# Autodesk Inventor assembly: electronics
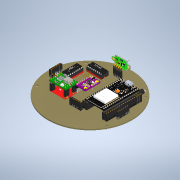
[picture p0: Inventor's stored thumbnail of the model, 180x180]
Saved by Autodesk Inventor 2020.2 (Build 242310000, 310)
## iProperties
Created: 2020-06-15
Part Number: electronics
Document SubType Name: Assembly
Designer: Tarsoly
Author: Tarsoly
## Documents named in this file (16)
- D:\Users\Tarsoly\Dokumentumok\BME\8. Félév\Önlab\3d\electronics.iam
- D:\Users\Tarsoly\Dokumentumok\BME\8. Félév\Önlab\3d\pins\socket\10x1\FH01-10SS.iam
- D:\Users\Tarsoly\Dokumentumok\BME\8. Félév\Önlab\3d\pins\socket\9x1\FH01-09SS.iam
- D:\Users\Tarsoly\Dokumentumok\BME\8. Félév\Önlab\3d\ESP32\ESP32S Dev Board 0.9inch width ASSY_TOP.iam
- D:\Users\Tarsoly\Dokumentumok\BME\8. Félév\Önlab\3d\PCB_v2\main_board.iam
- D:\Users\Tarsoly\Dokumentumok\BME\8. Félév\Önlab\3d\pins\socket\6x1\FH01-06SS.iam
- D:\Users\Tarsoly\Dokumentumok\BME\8. Félév\Önlab\3d\pins\dip_socket\IC_Sockel_16P.ipt
- D:\Users\Tarsoly\Dokumentumok\BME\8. Félév\Önlab\3d\L293D\L293D v1.iam
- D:\Users\Tarsoly\Dokumentumok\BME\8. Félév\Önlab\3d\pins\socket\4x1\FH01-04SS.iam
- D:\Users\Tarsoly\Dokumentumok\BME\8. Félév\Önlab\3d\pins\socket\3x1\FH01-03SS.iam
- D:\Users\Tarsoly\Dokumentumok\BME\8. Félév\Önlab\3d\pins\socket\2x1\FH01-02SS.iam
- D:\Users\Tarsoly\Dokumentumok\BME\8. Félév\Önlab\3d\pins\header\Pin Header 1x2 TH Pitch 2.54mm.ipt
- D:\Users\Tarsoly\Dokumentumok\BME\8. Félév\Önlab\3d\pins\header\Pin Header 1x4 TH Angle Pitch 2.54mm.ipt
- D:\Users\Tarsoly\Dokumentumok\BME\8. Félév\Önlab\3d\MPU2950\GY-91.iam
- D:\Users\Tarsoly\Dokumentumok\BME\8. Félév\Önlab\3d\VL5310X\vl53l0x.ipt
- D:\Users\Tarsoly\Dokumentumok\BME\8. Félév\Önlab\3d\DSN-1504\DC-DC 4.5-28V to 0.8-20V Output 3A MP1584EN Step Down Buck Converter_TOP.iam
## Components (32 placed, 15 different names)
1. FH01-10SS:1 [sub-assembly]
2. FH01-10SS:2 [sub-assembly]
3. FH01-09SS:1 [sub-assembly]
4. FH01-09SS:2 [sub-assembly]
5. ESP32S Dev Board 0.9inch width ASSY_TOP:1 [sub-assembly]
6. main_board:1 [sub-assembly]
7. FH01-10SS:3 [sub-assembly]
8. FH01-09SS:3 [sub-assembly]
9. FH01-10SS:4 [sub-assembly]
10. FH01-09SS:4 [sub-assembly]
11. FH01-06SS:1 [sub-assembly]
12. FH01-06SS:2 [sub-assembly]
13. FH01-06SS:3 [sub-assembly]
14. IC_Sockel_16P:1
15. IC_Sockel_16P:2
16. L293D v1:1 [sub-assembly]
17. L293D v1:2 [sub-assembly]
18. FH01-04SS:1 [sub-assembly]
19. FH01-04SS:2 [sub-assembly]
20. FH01-03SS:1 [sub-assembly]
21. FH01-02SS:1 [sub-assembly]
22. FH01-02SS:2 [sub-assembly]
23. Pin Header 1x2 TH Pitch 2.54mm:1
24. Pin Header 1x2 TH Pitch 2.54mm:2
25. Pin Header 1x4 TH Angle Pitch 2.54mm:1
26. FH01-02SS:3 [sub-assembly]
27. FH01-02SS:4 [sub-assembly]
28. GY-91:1 [sub-assembly]
29. vl53l0x:1
30. DC-DC 4.5-28V to 0.8-20V Output 3A MP1584EN Step Down Buck Converter_TOP:1 [sub-assembly]
31. Pin Header 1x2 TH Pitch 2.54mm:3
32. Pin Header 1x2 TH Pitch 2.54mm:4
## Relationships (87: Mate 77, Flush 8, Angle 2)
- [Mate]: FH01-09SS:1 ↔ ESP32S Dev Board 0.9inch width ASSY_TOP:1
- [Flush]: FH01-09SS:2 ↔ ESP32S Dev Board 0.9inch width ASSY_TOP:1
- [Flush]: FH01-09SS:2 ↔ ESP32S Dev Board 0.9inch width ASSY_TOP:1
- [Mate]: FH01-09SS:1 ↔ main_board:1
- [Mate]: FH01-09SS:1 ↔ main_board:1
- [Mate]: FH01-10SS:1 ↔ main_board:1
- [Mate]: FH01-10SS:1 ↔ main_board:1
- [Mate]: FH01-09SS:2 ↔ main_board:1
- [Mate]: FH01-09SS:2 ↔ main_board:1
- [Mate]: FH01-10SS:2 ↔ main_board:1
- [Mate]: FH01-10SS:2 ↔ main_board:1
- [Mate]: main_board:1 ↔ FH01-10SS:3
- [Mate]: main_board:1 ↔ FH01-10SS:3
- [Mate]: main_board:1 ↔ FH01-10SS:3
- [Mate]: main_board:1 ↔ FH01-09SS:3
- [Mate]: main_board:1 ↔ FH01-09SS:3
- [Mate]: main_board:1 ↔ FH01-09SS:3
- [Mate]: main_board:1 ↔ FH01-09SS:4
- [Mate]: main_board:1 ↔ FH01-09SS:4
- [Mate]: main_board:1 ↔ FH01-09SS:4
- [Mate]: main_board:1 ↔ FH01-10SS:4
- [Mate]: main_board:1 ↔ FH01-10SS:4
- [Mate]: main_board:1 ↔ FH01-10SS:4
- [Mate]: main_board:1 ↔ FH01-06SS:1
- [Mate]: main_board:1 ↔ FH01-06SS:1
- [Mate]: main_board:1 ↔ FH01-06SS:1
- [Mate]: main_board:1 ↔ FH01-06SS:2
- [Mate]: main_board:1 ↔ FH01-06SS:2
- [Mate]: main_board:1 ↔ FH01-06SS:2
- [Mate]: main_board:1 ↔ FH01-06SS:3
- [Mate]: main_board:1 ↔ FH01-06SS:3
- [Mate]: main_board:1 ↔ FH01-06SS:3
- [Mate]: main_board:1 ↔ IC_Sockel_16P:1
- [Mate]: main_board:1 ↔ IC_Sockel_16P:1
- [Mate]: main_board:1 ↔ IC_Sockel_16P:1
- [Mate]: main_board:1 ↔ IC_Sockel_16P:2
- [Mate]: main_board:1 ↔ IC_Sockel_16P:2
- [Mate]: main_board:1 ↔ IC_Sockel_16P:2
- [Mate]: IC_Sockel_16P:1 ↔ L293D v1:1
- [Mate]: IC_Sockel_16P:1 ↔ L293D v1:1
- [Mate] (-1.522 mm): IC_Sockel_16P:1 ↔ L293D v1:1
- [Mate]: IC_Sockel_16P:2 ↔ L293D v1:2
- [Mate]: IC_Sockel_16P:2 ↔ L293D v1:2
- [Mate] (-1.518 mm): IC_Sockel_16P:2 ↔ L293D v1:2
- [Mate]: main_board:1 ↔ FH01-04SS:1
- [Mate]: main_board:1 ↔ FH01-04SS:1
- [Mate]: main_board:1 ↔ FH01-04SS:1
- [Mate]: main_board:1 ↔ FH01-04SS:2
- [Mate]: main_board:1 ↔ FH01-04SS:2
- [Mate]: main_board:1 ↔ FH01-04SS:2
- [Mate]: main_board:1 ↔ FH01-03SS:1
- [Mate]: main_board:1 ↔ FH01-03SS:1
- [Mate]: main_board:1 ↔ FH01-03SS:1
- [Mate]: main_board:1 ↔ FH01-02SS:2
- [Mate]: main_board:1 ↔ FH01-02SS:1
- [Mate]: main_board:1 ↔ FH01-02SS:1
- [Mate]: main_board:1 ↔ FH01-02SS:1
- [Mate]: main_board:1 ↔ FH01-02SS:2
- [Mate]: main_board:1 ↔ FH01-02SS:2
- [Mate]: main_board:1 ↔ Pin Header 1x2 TH Pitch 2.54mm:2
- [Mate]: main_board:1 ↔ Pin Header 1x2 TH Pitch 2.54mm:1
- [Mate]: main_board:1 ↔ Pin Header 1x2 TH Pitch 2.54mm:2
- [Mate]: main_board:1 ↔ Pin Header 1x2 TH Pitch 2.54mm:1
- [Mate]: FH01-04SS:1 ↔ Pin Header 1x4 TH Angle Pitch 2.54mm:1
- [Mate]: FH01-04SS:1 ↔ Pin Header 1x4 TH Angle Pitch 2.54mm:1
- [Angle] (180 deg): FH01-04SS:1 ↔ Pin Header 1x4 TH Angle Pitch 2.54mm:1
- [Mate]: FH01-04SS:2 ↔ GY-91:1
- [Flush]: FH01-04SS:2 ↔ GY-91:1
- [Flush]: FH01-04SS:2 ↔ GY-91:1
- [Mate]: Pin Header 1x4 TH Angle Pitch 2.54mm:1 ↔ vl53l0x:1
- [Mate]: Pin Header 1x4 TH Angle Pitch 2.54mm:1 ↔ vl53l0x:1
- [Mate] (11.12 mm): main_board:1 ↔ vl53l0x:1
- [Mate]: FH01-02SS:4 ↔ DC-DC 4.5-28V to 0.8-20V Output 3A MP1584EN Step Down Buck Converter_TOP:1
- [Mate]: FH01-02SS:3 ↔ DC-DC 4.5-28V to 0.8-20V Output 3A MP1584EN Step Down Buck Converter_TOP:1
- [Mate]: FH01-02SS:4 ↔ DC-DC 4.5-28V to 0.8-20V Output 3A MP1584EN Step Down Buck Converter_TOP:1
- [Mate]: FH01-02SS:3 ↔ DC-DC 4.5-28V to 0.8-20V Output 3A MP1584EN Step Down Buck Converter_TOP:1
- [Flush] (0.55 mm): FH01-02SS:3 ↔ DC-DC 4.5-28V to 0.8-20V Output 3A MP1584EN Step Down Buck Converter_TOP:1
- [Flush] (0.55 mm): FH01-02SS:4 ↔ DC-DC 4.5-28V to 0.8-20V Output 3A MP1584EN Step Down Buck Converter_TOP:1
- [Mate]: DC-DC 4.5-28V to 0.8-20V Output 3A MP1584EN Step Down Buck Converter_TOP:1 ↔ Pin Header 1x2 TH Pitch 2.54mm:3
- [Mate]: DC-DC 4.5-28V to 0.8-20V Output 3A MP1584EN Step Down Buck Converter_TOP:1 ↔ Pin Header 1x2 TH Pitch 2.54mm:4
- [Mate]: DC-DC 4.5-28V to 0.8-20V Output 3A MP1584EN Step Down Buck Converter_TOP:1 ↔ Pin Header 1x2 TH Pitch 2.54mm:4
- [Mate]: DC-DC 4.5-28V to 0.8-20V Output 3A MP1584EN Step Down Buck Converter_TOP:1 ↔ Pin Header 1x2 TH Pitch 2.54mm:3
- [Flush] (0.53 mm): DC-DC 4.5-28V to 0.8-20V Output 3A MP1584EN Step Down Buck Converter_TOP:1 ↔ Pin Header 1x2 TH Pitch 2.54mm:3
- [Flush] (0.53 mm): DC-DC 4.5-28V to 0.8-20V Output 3A MP1584EN Step Down Buck Converter_TOP:1 ↔ Pin Header 1x2 TH Pitch 2.54mm:4
- [Mate]: FH01-02SS:2 ↔ Pin Header 1x2 TH Pitch 2.54mm:4
- [Mate]: FH01-02SS:2 ↔ Pin Header 1x2 TH Pitch 2.54mm:3
- [Angle] (180 deg): FH01-02SS:2 ↔ Pin Header 1x2 TH Pitch 2.54mm:4
## Named parameters: d70_d71 = 0 mm, d71_d72 = 0 mm, d72_d73 = 0 mm, d73_d74 = 0 mm, d74_d75 = 0 mm, d75_d76 = 0 mm, d76_d77 = 0 mm, d77_d78 = 0 mm, d78_d79 = 0 mm, d79_d80 = 0 mm, d80_d81 = 0 mm, d81_d82 = 0 mm, d82_d83 = 0 mm, d83_d84 = 0 mm, d84_d85 = 0 mm, d85_d86 = 0 mm
